# Autodesk Inventor assembly: SHHPSK5-2
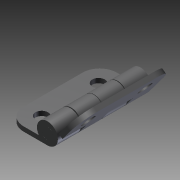
[picture p0: Inventor's stored thumbnail of the model, 180x180]
Saved by Autodesk Inventor 2015 SP1 (Build 190203100, 203)
## iProperties
Category: Hardware
Company: MISUMI
Created: 2015-01-26
Part Number: SHHPSK5-2
Catalog Web Link: http://us.misumi-ec.com/vona2/detail/110302361830/
Description: SHHPS, SHHPT, SHHPSK-Stainless Steel Hinges, Steel Hinges
Vendor: MISUMI
Document SubType Name: Assembly
Designer: PARTuser1
Manufacturer: MISUMI
Stock Number: SHHPSK5-2
PSOL_IDENT_0: {\\10.0.0.236\data_v8\23d-libs\misumi\metric\39_accessories_for_al_extrusions\shhpt_asmtab.prj},194
PSOL_IDENT_1: {VTYP=3D},{STYP=ASSTAB},{NB=SHHPSK5-2},{LINA=SHHPSK5-2},{NN=SHHPS, SHHPT, SHHPSK},{DATE=17.11.2014 0
PSOL_IDENT_2: 5:31:35},{GEOMDATE=29.04.2010},{VERSION=},{LINEID=10},{LINESUBID=-1},{WBVAR=TS,MAT,NOH,ALT1}  {NB=SH
PSOL_IDENT_3: HPSK5-2},{LINA=SHHPSK5-2},{KT=DUMMY},{PN=SHHPSK5-2},{TYPE=SHHPSK},{TS=1},{MAT=304},{MATALG= '316','3
PSOL_IDENT_4: 16 Stainless Steel','304','304 Stainless Steel' },{ST=Satin Finish},{NO=5},{NOH=2},{ALKG=9},{ALN=88}
PSOL_IDENT_5: ,{MASS=43},{L=41},{W=36},{K=8.0},{P=25},{J=7.5},{S=21},{N=5.5},{T=2.0},{E=4.6},{R=4.6},{CR=7.5},{D=5
PSOL_IDENT_6: },{AB=CBSST5-8},{QB=4},{AN=HNTTSN5-5},{QN=4},{ALT1=},{TIF=1},{PPATH=shhps_asmtpl.prj}
SUPPLIER: MISUMI
ARTICLENO: SHHPSK5-2
BOMINFO: SHHPSK5-2
CREATOR: CADENAS GmbH
Title: Hinge
Author: Misumi
## Documents named in this file (4)
- C:\Users\Jack\ownCloud\Projects\CrossBot\InventorModel\Hardware\Hinges\HingeSHHPSK5-2\SHHPSK5_2.iam
- C:\Users\Jack\ownCloud\Projects\CrossBot\InventorModel\Hardware\Hinges\HingeSHHPSK5-2\SHHPS5_2_r.ipt
- C:\Users\Jack\ownCloud\Projects\CrossBot\InventorModel\Hardware\Hinges\HingeSHHPSK5-2\SHHPS5_2_pin.ipt
- C:\Users\Jack\ownCloud\Projects\CrossBot\InventorModel\Hardware\Hinges\HingeSHHPSK5-2\SHHPS5_2_l.ipt
## Components (3 placed, 3 different names)
1. SHHPS5_2_r:1 — Mate:1, Flush:1
2. SHHPS5_2_pin:1 — Mate:1, Flush:1
3. SHHPS5_2_l:1
## Relationships (2: Mate 1, Flush 1)
- Mate:1: SHHPS5_2_r:1 ↔ SHHPS5_2_pin:1
- Flush:1: SHHPS5_2_r:1 ↔ SHHPS5_2_pin:1
